# Autodesk Inventor assembly: Idler Assembly
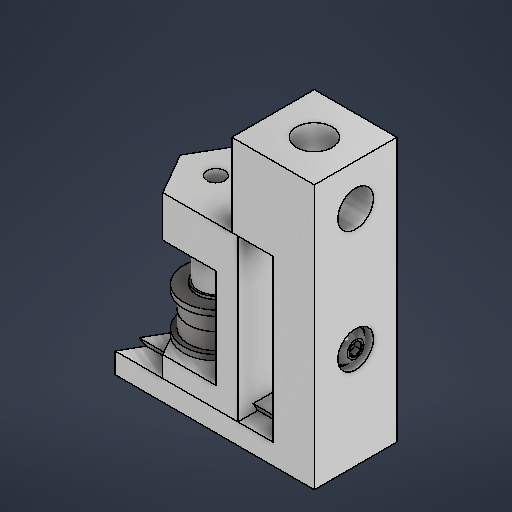
[picture p0: Inventor's stored thumbnail of the model, 512x512]
Saved by Autodesk Inventor 2026 (Build 300175050, 175E)
## iProperties
Created: 2025-05-27
Part Number: Idler Assembly
Document SubType Name: Assembly
Designer: Joshua Eah
Author: Joshua Eah
## Documents named in this file (4)
- C:\Users\Joshua Eah\Documents\GitHub\Voron-0\CAD\Tulip - Machined Parts\Idlers\Idler Assembly.iam
- C:\Users\Joshua Eah\Documents\GitHub\Voron-0\CAD\Tulip - Machined Parts\Idlers\A Idler (Tulip).ipt
- C:\Users\Joshua Eah\Documents\GitHub\Voron-0\CAD\Tulip - Machined Parts\Idlers\Bearing Sled.iam
- C:\Users\Joshua Eah\Documents\GitHub\Voron-0\CAD\Master Assembly\Hardware\M3x12 BHCS.ipt
## Components (3 placed, 3 different names)
1. A Idler (Tulip):1 — Mate:1, Flush:1, Insert:1, Flush:2
2. Bearing Sled:1 [sub-assembly] — Mate:1, Flush:1, Flush:2
3. M3x12 BHCS:1 — Insert:1
## Relationships (4: Flush 2, Mate 1, Insert 1)
- Mate:1: A Idler (Tulip):1 ↔ Bearing Sled:1
- Flush:1: A Idler (Tulip):1 ↔ Bearing Sled:1
- Insert:1: A Idler (Tulip):1 ↔ M3x12 BHCS:1
- Flush:2: A Idler (Tulip):1 ↔ Bearing Sled:1
